# Autodesk Inventor assembly: Confirmat Joint1101
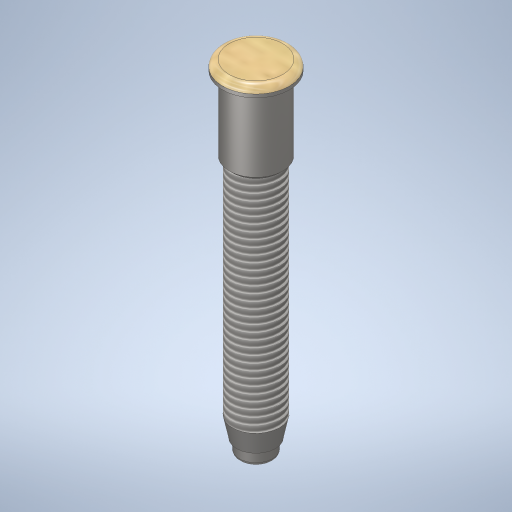
[picture p0: Inventor's stored thumbnail of the model, 512x512]
Saved by Autodesk Inventor 2024 (Build 280153000, 153)
## iProperties
RuleStatus: InUse
Created: 2021-09-13
Part Number: Confirmat Joint1101
Document SubType Name: Assembly
Designer: RokasM
Author: RokasM
## Documents named in this file (3)
- C:\W4INV 2024 Design\PROJECTS\Samples\Macro DEMO\7 Computer Case\Computer Case.iam Smart Hardware\Confirmat Joint11\Confirmat Joint1101.iam
- C:\W4INV 2024 Design\PROJECTS\MODEL STATE LIBRARY COMPONENTS\Confirmat\Cap.ipt
- C:\W4INV 2024 Design\PROJECTS\Samples\Macro DEMO\7 Computer Case\Computer Case.iam Smart Hardware\Confirmat Joint11\Confirmat Joint110100.ipt
## Components (2 placed, 2 different names)
1. Confirmat
2. Cap — Flush:1
## Relationships (1: Flush 1)
- Flush:1: Cap
## Named parameters: Nestled_Board_Thickness = 18 mm
